# Autodesk Inventor assembly: Base 8020
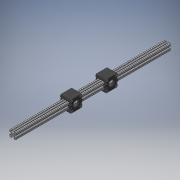
[picture p0: Inventor's stored thumbnail of the model, 180x180]
Saved by Autodesk Inventor 2018 (Build 220112000, 112)
## iProperties
Created: 2020-01-31
Part Number: Base 8020
Document SubType Name: Assembly
Designer: Weeb No1
Author: Weeb No1
## Documents named in this file (3)
- C:\Users\Weeb No1\Documents\GitHub\2020CAD\Gabriel Inventor Files (Shooter, Drivebase)\Drivebase Assembly\Base 8020.iam
- C:\Users\Weeb No1\Documents\GitHub\2020CAD\Gabriel Inventor Files (Shooter, Drivebase)\Drivebase Assembly\Part Files\8020 1010 x 19 v2.ipt
- C:\Users\Weeb No1\Documents\GitHub\2020CAD\Gabriel Inventor Files (Shooter, Drivebase)\Drivebase Assembly\Part Files\VersaBlock_Mini_Kit_217-5852.iam
## Components (3 placed, 2 different names)
1. 8020 1010 x 19 v2:1 — Mate:1, Mate:2, Mate:3, Mate:4
2. VersaBlock_Mini_Kit_217-5852:1 [sub-assembly] — Mate:1, Mate:2
3. VersaBlock_Mini_Kit_217-5852:2 [sub-assembly] — Mate:3, Mate:4
## Relationships (4: Mate 4)
- Mate:1: 8020 1010 x 19 v2:1 ↔ VersaBlock_Mini_Kit_217-5852:1
- Mate:2: 8020 1010 x 19 v2:1 ↔ VersaBlock_Mini_Kit_217-5852:1
- Mate:3: 8020 1010 x 19 v2:1 ↔ VersaBlock_Mini_Kit_217-5852:2
- Mate:4: 8020 1010 x 19 v2:1 ↔ VersaBlock_Mini_Kit_217-5852:2
